# Autodesk Inventor assembly: pcb_assembly
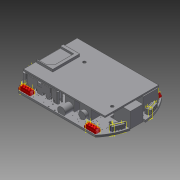
[picture p0: Inventor's stored thumbnail of the model, 180x180]
Saved by Autodesk Inventor 2014 (Build 180170000, 170)
## iProperties
Created: 2013-08-25
Part Number: pcb_assembly
Document SubType Name: Assembly
Designer: Felix
Author: Felix
## Documents named in this file (3)
- C:\Users\Felix\Desktop\Beep\Hardware\3D-CAD\electronic\pcb_assembly.iam
- C:\Users\Felix\Desktop\Beep\Hardware\3D-CAD\electronic\BEEP\beep_main_assembled.iam
- C:\Users\Felix\Desktop\Beep\Hardware\3D-CAD\electronic\RaspberryPi\RaspberryPi.iam
## Components (2 placed, 2 different names)
1. beep_main_assembled:1 [sub-assembly] — Passend:2
2. RaspberryPi:1 [sub-assembly] — Passend:2
## Relationships (1: Mate 1)
- Passend:2 [Mate]: beep_main_assembled:1 ↔ RaspberryPi:1
